# Autodesk Inventor assembly: МПСТ Редуктор
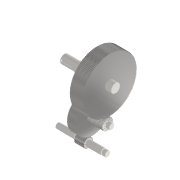
[picture p0: Inventor's stored thumbnail of the model, 180x180]
Saved by Autodesk Inventor 2022 (Build 260153000, 153)
## iProperties
Created: 2021-09-16
Part Number: МПСТ Редуктор
Document SubType Name: Assembly
Designer: Алексанян Г.
Author: Алексанян Г.
## Documents named in this file (6)
- C:\Учёба\5 семестр\Дет. Маш\Редуктор (копия для расчетов)\МПСТ Редуктор.iam
- C:\Учёба\5 семестр\Дет. Маш\Редуктор (копия для расчетов)\МПСТ Промежуточный Вал.iam
- C:\Учёба\5 семестр\Дет. Маш\Редуктор (копия для расчетов)\МПСТ Тихоходный Вал.iam
- C:\Учёба\5 семестр\Дет. Маш\Редуктор (копия для расчетов)\МПСТ Редуктор\Мастер проектирования\Цилиндрическое зубчатое зацепление1.iam
- C:\Учёба\5 семестр\Дет. Маш\Редуктор (копия для расчетов)\МПСТ Быстроходный Вал.iam
- C:\Учёба\5 семестр\Дет. Маш\Редуктор (копия для расчетов)\МПСТ Редуктор\Мастер проектирования\Цилиндрическое зубчатое зацепление2.iam
## Components (5 placed, 4 different names)
1. МПСТ Промежуточный Вал:1 [sub-assembly] — Угол:1, Совмещение:1, Совмещение:5, Совмещение:15, Заподлицо:5, Совмещение:19, Совмещение:20
2. МПСТ Тихоходный Вал:1 [sub-assembly] — Угол:1, Совмещение:1, Совмещение:16, Совмещение:17
3. Цилиндрическое зубчатое зацепление:1 [sub-assembly] — Совмещение:15, Заподлицо:5, Совмещение:16, Совмещение:17
4. МПСТ Быстроходный Вал:1 [sub-assembly] — Совмещение:5, Совмещение:18, Заподлицо:6
5. Цилиндрическое зубчатое зацепление:2 [sub-assembly] — Совмещение:18, Заподлицо:6, Совмещение:19, Совмещение:20
## Relationships (11: Mate 8, Flush 2, Angle 1)
- Угол:1 [Angle] (0 deg): МПСТ Промежуточный Вал:1 ↔ МПСТ Тихоходный Вал:1
- Совмещение:1 [Mate] (300 mm): МПСТ Промежуточный Вал:1 ↔ МПСТ Тихоходный Вал:1
- Совмещение:5 [Mate] (200 mm): МПСТ Промежуточный Вал:1 ↔ МПСТ Быстроходный Вал:1
- Совмещение:15 [Mate]: МПСТ Промежуточный Вал:1 ↔ Цилиндрическое зубчатое зацепление:1
- Заподлицо:5 [Flush]: МПСТ Промежуточный Вал:1 ↔ Цилиндрическое зубчатое зацепление:1
- Совмещение:16 [Mate]: МПСТ Тихоходный Вал:1 ↔ Цилиндрическое зубчатое зацепление:1
- Совмещение:17 [Mate]: МПСТ Тихоходный Вал:1 ↔ Цилиндрическое зубчатое зацепление:1
- Совмещение:18 [Mate]: МПСТ Быстроходный Вал:1 ↔ Цилиндрическое зубчатое зацепление:2
- Заподлицо:6 [Flush]: МПСТ Быстроходный Вал:1 ↔ Цилиндрическое зубчатое зацепление:2
- Совмещение:19 [Mate]: МПСТ Промежуточный Вал:1 ↔ Цилиндрическое зубчатое зацепление:2
- Совмещение:20 [Mate]: МПСТ Промежуточный Вал:1 ↔ Цилиндрическое зубчатое зацепление:2
